# Autodesk Inventor assembly: Glock Assembly
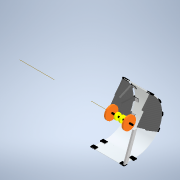
[picture p0: Inventor's stored thumbnail of the model, 180x180]
Saved by Autodesk Inventor 2020 (Build 240168000, 168)
## iProperties
Created: 2021-01-17
Part Number: Glock Assembly
Document SubType Name: Assembly
Designer: magda
Author: magda
## Documents named in this file (8)
- C:\Users\magda\OneDrive\Documents\Inventor\T3\Glock\Glock Assembly.iam
- C:\Users\magda\OneDrive\Documents\Inventor\T3\Glock\Shaft.ipt
- C:\Users\magda\OneDrive\Documents\Inventor\T3\Glock\2 in Compliance Wheel.ipt
- C:\Users\magda\OneDrive\Documents\Inventor\T3\Glock\4 in Compliance Wheel.ipt
- C:\Users\magda\OneDrive\Documents\Inventor\T3\Glock\External Lexan.ipt
- C:\Users\magda\OneDrive\Documents\Inventor\T3\Glock\Shield Assembly.iam
- C:\Users\magda\OneDrive\Documents\Inventor\T3\Glock\Flat Fastener.ipt
- C:\Users\magda\OneDrive\Documents\Inventor\T3\Glock\Support Bracket 1.ipt
## Components (12 placed, 7 different names)
1. Shaft:1 — Mate:1, Mate:2, Mate:3, Mate:4, Flush:1, Flush:2, Flush:3, Flush:4, Mate:6, Flush:6
2. 2 in Compliance Wheel:1 — Mate:1, Flush:4
3. 2 in Compliance Wheel:2 — Mate:2, Flush:3
4. 4 in Compliance Wheel:1 — Mate:4, Flush:2
5. 4 in Compliance Wheel:2 — Mate:3, Flush:1
6. External Lexan:1 — Flush:6, Mate:7, Mate:10, Mate:11, Flush:7, Mate:12, Mate:13, Mate:14, Mate:15, Mate:16, Flush:8, Mate:17, Mate:18, Mate:19, Mate:20
7. Shield Assembly:1 [sub-assembly] — Mate:9
8. Flat Fastener:1 — Mate:11, Flush:7, Mate:12, Flush:9, Mate:21, Flush:10
9. Flat Fastener:2 — Mate:18, Mate:19, Mate:20
10. Flat Fastener:3 — Mate:13, Mate:14, Mate:15
11. Flat Fastener:4 — Mate:16, Flush:8, Mate:17
12. Support Bracket 1:1 — Flush:9, Mate:21, Flush:10
## Relationships (29: Mate 20, Flush 9)
- Mate:1: Shaft:1 ↔ 2 in Compliance Wheel:1
- Mate:2: Shaft:1 ↔ 2 in Compliance Wheel:2
- Mate:3: Shaft:1 ↔ 4 in Compliance Wheel:2
- Mate:4: Shaft:1 ↔ 4 in Compliance Wheel:1
- Flush:1 (25.4 mm): Shaft:1 ↔ 4 in Compliance Wheel:2
- Flush:2 (25.4 mm): Shaft:1 ↔ 4 in Compliance Wheel:1
- Flush:3 (76.2 mm): Shaft:1 ↔ 2 in Compliance Wheel:2
- Flush:4 (76.2 mm): Shaft:1 ↔ 2 in Compliance Wheel:1
- Mate:6: Shaft:1
- Flush:6 (19.05 mm): Shaft:1 ↔ External Lexan:1
- Mate:7: External Lexan:1
- Mate:8
- Mate:9: Shield Assembly:1
- Mate:10: External Lexan:1
- Mate:11: External Lexan:1 ↔ Flat Fastener:1
- Flush:7: External Lexan:1 ↔ Flat Fastener:1
- Mate:12: External Lexan:1 ↔ Flat Fastener:1
- Mate:13: External Lexan:1 ↔ Flat Fastener:3
- Mate:14: External Lexan:1 ↔ Flat Fastener:3
- Mate:15: External Lexan:1 ↔ Flat Fastener:3
- Mate:16: External Lexan:1 ↔ Flat Fastener:4
- Flush:8: External Lexan:1 ↔ Flat Fastener:4
- Mate:17: External Lexan:1 ↔ Flat Fastener:4
- Mate:18: External Lexan:1 ↔ Flat Fastener:2
- Mate:19: External Lexan:1 ↔ Flat Fastener:2
- Mate:20: External Lexan:1 ↔ Flat Fastener:2
- Flush:9: Flat Fastener:1 ↔ Support Bracket 1:1
- Mate:21: Flat Fastener:1 ↔ Support Bracket 1:1
- Flush:10: Flat Fastener:1 ↔ Support Bracket 1:1
